# Autodesk Inventor assembly: PowerDetector
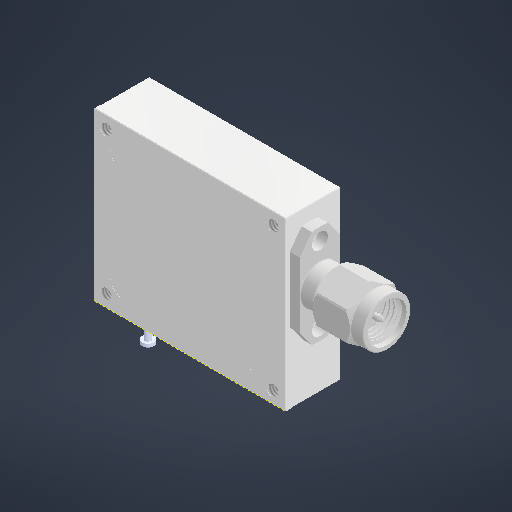
[picture p0: Inventor's stored thumbnail of the model, 512x512]
Saved by Autodesk Inventor 2026.2 (Build 302298010, 298A)
## iProperties
Created: 2026-06-22
Part Number: PowerDetector
Document SubType Name: Assembly
Designer: sonata
Author: sonata
## Documents named in this file (5)
- Z:\crush\mechanical\PAM-modules-mount\PowerDetector.iam
- Z:\crush\Front-Page\Analog-Signal-Components\PAX\PAM-2025\PAM-modules\detector-module\detector-module-v2\enclosure\Detector Box ND20.ipt
- Z:\crush\Front-Page\Analog-Signal-Components\PAX\PAM-2025\PAM-modules\detector-module\detector-module-v2\enclosure\Detector Lid ND20.ipt
- Z:\crush\mechanical\PAM-modules-mount\PE44032_3D\PE44032_3D\PE44032_3D.ipt
- Z:\crush\mechanical\PAM-modules-mount\1595-2\1595-2\1595-2.ipt
## Components (4 placed, 4 different names)
1. Detector Box ND20:1 — Mate:1, Mate:2, Mate:3, Mate:4
2. Detector Lid ND20:1 — Mate:1, Mate:4, Flush:1
3. PE44032_3D:1 — Mate:2
4. 1595-2:1 — Mate:3, Flush:1
## Relationships (5: Mate 4, Flush 1)
- Mate:1: Detector Box ND20:1 ↔ Detector Lid ND20:1
- Mate:2: Detector Box ND20:1 ↔ PE44032_3D:1
- Mate:3: Detector Box ND20:1 ↔ 1595-2:1
- Mate:4: Detector Box ND20:1 ↔ Detector Lid ND20:1
- Flush:1 (1.5 mm): Detector Lid ND20:1 ↔ 1595-2:1
